# Autodesk Inventor assembly: Bumper Assembly
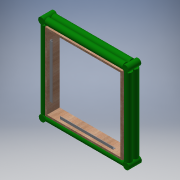
[picture p0: Inventor's stored thumbnail of the model, 180x180]
Saved by Autodesk Inventor 2018 (Build 220112000, 112)
## iProperties
Created: 2019-02-24
Part Number: Bumper Assembly
Document SubType Name: Assembly
Designer: maste
Author: maste
## Documents named in this file (3)
- C:\Users\maste\OneDrive\Documents\GitHub\2019CAD\Drivebase but Calvin is a mad man\Bumper Assembly.iam
- C:\Users\maste\OneDrive\Documents\GitHub\2019CAD\Drivebase but Calvin is a mad man\Bumper Side.ipt
- C:\Users\maste\OneDrive\Documents\GitHub\2019CAD\Drivebase but Calvin is a mad man\Bumper L.ipt
## Components (8 placed, 2 different names)
1. Bumper Side:1 — Mate:1, Flush:1, Flush:2, Mate:10, Mate:11, Mate:12
2. Bumper Side:2 — Mate:1, Flush:1, Flush:2, Flush:3, Flush:4, Mate:2, Mate:13, Mate:14, Mate:15
3. Bumper Side:3 — Flush:3, Flush:4, Mate:2, Flush:5, Flush:6, Mate:3, Mate:7, Mate:8, Mate:9
4. Bumper Side:4 — Flush:5, Flush:6, Mate:3, Mate:4, Mate:5, Mate:6
5. Bumper L:1 — Mate:4, Mate:5, Mate:6
6. Bumper L:2 — Mate:7, Mate:8, Mate:9
7. Bumper L:3 — Mate:13, Mate:14, Mate:15
8. Bumper L:4 — Mate:10, Mate:11, Mate:12
## Relationships (21: Mate 15, Flush 6)
- Mate:1: Bumper Side:1 ↔ Bumper Side:2
- Flush:1: Bumper Side:1 ↔ Bumper Side:2
- Flush:2: Bumper Side:1 ↔ Bumper Side:2
- Flush:3: Bumper Side:2 ↔ Bumper Side:3
- Flush:4: Bumper Side:2 ↔ Bumper Side:3
- Mate:2: Bumper Side:2 ↔ Bumper Side:3
- Flush:5: Bumper Side:3 ↔ Bumper Side:4
- Flush:6: Bumper Side:3 ↔ Bumper Side:4
- Mate:3: Bumper Side:3 ↔ Bumper Side:4
- Mate:4: Bumper Side:4 ↔ Bumper L:1
- Mate:5: Bumper Side:4 ↔ Bumper L:1
- Mate:6: Bumper Side:4 ↔ Bumper L:1
- Mate:7: Bumper Side:3 ↔ Bumper L:2
- Mate:8: Bumper Side:3 ↔ Bumper L:2
- Mate:9: Bumper Side:3 ↔ Bumper L:2
- Mate:10: Bumper Side:1 ↔ Bumper L:4
- Mate:11: Bumper Side:1 ↔ Bumper L:4
- Mate:12: Bumper Side:1 ↔ Bumper L:4
- Mate:13: Bumper Side:2 ↔ Bumper L:3
- Mate:14: Bumper Side:2 ↔ Bumper L:3
- Mate:15: Bumper Side:2 ↔ Bumper L:3
